# Autodesk Inventor assembly: BashyWingtip
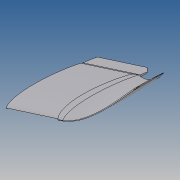
[picture p0: Inventor's stored thumbnail of the model, 180x180]
Saved by Autodesk Inventor 2019.4 (Build 234330000, 330)
## iProperties
Part Number: BashyWingtip
Document SubType Name: Assembly
Designer: Admin
Mass: 10567.1 g
Surface Area: 1636.4 cm^2
Volume: 1344.41 cm^3
Density: 7.86 g/cm^3
Author: Admin
Revision: -
VAULT_Status: in Bearbeitung
Gewicht: 10,567 kg
InventorVersion: 2019.4
## Documents named in this file (4)
- C:\Users\tonn\Documents\GitHub\CAD_Elements\STL\wing\BashyWingtip.iam
- Norm.iam
- C:\Users\tonn\Documents\GitHub\CAD_Elements\CAD\bashy\Wingtip.ipt
- C:\Users\tonn\Documents\GitHub\CAD_Elements\CAD\bashy\Wing_airfoil.ipt
## Components (2 placed, 2 different names)
1. WING_AIRFOIL_WINGTIP--IPT:1 — Fluchtend:1, Fluchtend:2, Passend:4
2. WING_AIRFOIL_WING_AIRFOIL--IPT:1 — Fluchtend:1, Fluchtend:2, Passend:4
## Relationships (3: Flush 2, Mate 1)
- Fluchtend:1 [Flush]: WING_AIRFOIL_WINGTIP--IPT:1 ↔ WING_AIRFOIL_WING_AIRFOIL--IPT:1
- Fluchtend:2 [Flush]: WING_AIRFOIL_WINGTIP--IPT:1 ↔ WING_AIRFOIL_WING_AIRFOIL--IPT:1
- Passend:4 [Mate] (1 mm): WING_AIRFOIL_WINGTIP--IPT:1 ↔ WING_AIRFOIL_WING_AIRFOIL--IPT:1
## Named parameters: Gewicht = 10.5671
note: some values were not read from the file. Shown as the stored number, unit unknown: "Gewicht".
